# Autodesk Inventor assembly: POM_T5_07
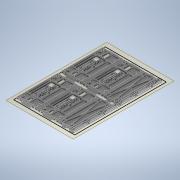
[picture p0: Inventor's stored thumbnail of the model, 180x180]
Saved by Autodesk Inventor 2022.3 (Build 263350000, 350)
## iProperties
Created: 2022-09-28
Part Number: POM_T5_07
Document SubType Name: Assembly
Designer: Masato
Author: Masato
## Documents named in this file (6)
- C:\Users\Masato\Documents\Inventor\Inventor for CIT Brains\SUSTAINA-OP\Cam\POM_T5\POM_T5_07.iam
- C:\Users\Masato\Documents\Inventor\Inventor for CIT Brains\SUSTAINA-OP\Cam\DisposableBoard.ipt
- C:\Users\Masato\Documents\Inventor\Inventor for CIT Brains\SUSTAINA-OP\UpperBody\Cockpit\Cockpit_back_frame.ipt
- C:\Users\Masato\Documents\Inventor\Inventor for CIT Brains\SUSTAINA-OP\OptionParts\DrillingJigs\Head_neck_diagonal_Jig_back.ipt
- C:\Users\Masato\Documents\Inventor\Inventor for CIT Brains\SUSTAINA-OP\OptionParts\DrillingJigs\Head_neck_diagonal_Jig_side.ipt
- C:\Users\Masato\Documents\Inventor\Inventor for CIT Brains\SUSTAINA-OP\UpperBody\Cockpit\Cockpit_battery_frame.ipt
## Components (25 placed, 5 different names)
1. DisposableBoard:1 — フラッシュ:1, フラッシュ:2, フラッシュ:3, フラッシュ:4, Flush:5, Flush:6
2. Head_neck_diagonal_Jig_side:9 — Mate:13, Mate:14, Flush:11
3. Cockpit_back_frame:1 — Mate:1, Flush:5, Flush:6, Mate:6, Mate:10
4. Head_neck_diagonal_Jig_side:1 — Mate:3, Flush:8, Mate:8, Flush:9, Mate:9
5. Head_neck_diagonal_Jig_side:2 — Mate:7, Mate:8, Flush:9
6. Head_neck_diagonal_Jig_back:1 — Mate:2, Mate:6, Flush:8, Mate:9, Mate:10
7. Cockpit_back_frame:2
8. Head_neck_diagonal_Jig_side:3
9. Head_neck_diagonal_Jig_side:6
10. Head_neck_diagonal_Jig_back:2
11. Cockpit_back_frame:3 — Flush:7, Mate:5
12. Head_neck_diagonal_Jig_side:4
13. Head_neck_diagonal_Jig_side:7
14. Head_neck_diagonal_Jig_back:3
15. Cockpit_back_frame:4
16. Head_neck_diagonal_Jig_side:5
17. Head_neck_diagonal_Jig_side:8
18. Head_neck_diagonal_Jig_back:4
19. Cockpit_battery_frame:1 — Mate:4, Flush:7, Mate:5, Flush:10, Mate:12
20. Cockpit_battery_frame:2
21. Head_neck_diagonal_Jig_back:5 — Mate:11, Flush:10, Mate:12
22. Head_neck_diagonal_Jig_back:6
23. Head_neck_diagonal_Jig_back:7
24. Head_neck_diagonal_Jig_back:8
25. Head_neck_diagonal_Jig_back:9 — Mate:14, Flush:11
## Component patterns: (4 elements, first: Cockpit_back_frame:1 + Head_neck_diagonal_Jig_side:1 + Head_neck_diagonal_Jig_side:2 + Head_neck_diagonal_Jig_back:1), (2 elements, first: Cockpit_battery_frame:1), (5 elements, first: Head_neck_diagonal_Jig_back:5)
## Relationships (25: Mate 14, Flush 11)
- フラッシュ:1 [Flush]: DisposableBoard:1
- フラッシュ:2 [Flush]: DisposableBoard:1
- フラッシュ:3 [Flush]: DisposableBoard:1
- フラッシュ:4 [Flush]: DisposableBoard:1
- Mate:1: Cockpit_back_frame:1
- Flush:5 (-2 mm): DisposableBoard:1 ↔ Cockpit_back_frame:1
- Flush:6 (-2 mm): DisposableBoard:1 ↔ Cockpit_back_frame:1
- Mate:2: Head_neck_diagonal_Jig_back:1
- Mate:3: Head_neck_diagonal_Jig_side:1
- Mate:4: Cockpit_battery_frame:1
- Flush:7: Cockpit_back_frame:3 ↔ Cockpit_battery_frame:1
- Mate:5 (2.1 mm): Cockpit_back_frame:3 ↔ Cockpit_battery_frame:1
- Mate:6 (4.5 mm): Cockpit_back_frame:1 ↔ Head_neck_diagonal_Jig_back:1
- Flush:8: Head_neck_diagonal_Jig_side:1 ↔ Head_neck_diagonal_Jig_back:1
- Mate:7: Head_neck_diagonal_Jig_side:2
- Mate:8 (2.1 mm): Head_neck_diagonal_Jig_side:1 ↔ Head_neck_diagonal_Jig_side:2
- Flush:9: Head_neck_diagonal_Jig_side:1 ↔ Head_neck_diagonal_Jig_side:2
- Mate:9 (2.1 mm): Head_neck_diagonal_Jig_side:1 ↔ Head_neck_diagonal_Jig_back:1
- Mate:10 (2.1 mm): Cockpit_back_frame:1 ↔ Head_neck_diagonal_Jig_back:1
- Mate:11: Head_neck_diagonal_Jig_back:5
- Flush:10: Cockpit_battery_frame:1 ↔ Head_neck_diagonal_Jig_back:5
- Mate:12 (2.1 mm): Cockpit_battery_frame:1 ↔ Head_neck_diagonal_Jig_back:5
- Mate:13: Head_neck_diagonal_Jig_side:9
- Mate:14 (2.1 mm): Head_neck_diagonal_Jig_side:9 ↔ Head_neck_diagonal_Jig_back:9
- Flush:11: Head_neck_diagonal_Jig_side:9 ↔ Head_neck_diagonal_Jig_back:9
